# Autodesk Inventor assembly: 0008-10-10 Injectomat Standard
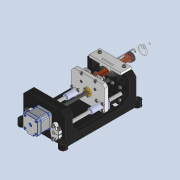
[picture p0: Inventor's stored thumbnail of the model, 180x180]
Saved by Autodesk Inventor 2020 (Build 240168000, 168)
## iProperties
Created: 2021-02-20
Part Number: 0008-10-10 Injectomat Standard
Document SubType Name: Assembly
Designer: Iulian Bors
Mass: 1274.49 g
Surface Area: 2683.15 cm^2
Volume: 830.675 cm^3
Density: 1.53428 g/cm^3
Description: Injectomat standard
Author: Iulian Bors
Subject: 10-10
## Documents named in this file (27)
- Z:\I.A.B\Proiecte\0008 I.A.B 3D 2.1 Imprimanta aracet Metal\10 Mecanic\0008-10-10 Injectomat Standard.iam
- Z:\I.A.B\Proiecte\0008 I.A.B 3D 2.1 Imprimanta aracet Metal\10 Mecanic\Seringa\syringe-57.snapshot.2\SYRINGE (INVENTOR)\Body Syringe.ipt
- Z:\I.A.B\Proiecte\0008 I.A.B 3D 2.1 Imprimanta aracet Metal\10 Mecanic\Seringa\syringe-57.snapshot.2\SYRINGE (INVENTOR)\Plunger.ipt
- Z:\I.A.B\Proiecte\0008 I.A.B 3D 2.1 Imprimanta aracet Metal\10 Mecanic\Seringa\syringe-57.snapshot.2\SYRINGE (INVENTOR)\Plunger Rubber.ipt
- Z:\I.A.B\Proiecte\0008 I.A.B 3D 2.1 Imprimanta aracet Metal\10 Mecanic\0008-10-1000 LMK8LUU.ipt
- Z:\I.A.B\Proiecte\0008 I.A.B 3D 2.1 Imprimanta aracet Metal\10 Mecanic\0008-10-1002  Hub.ipt
- Z:\I.A.B\Proiecte\0008 I.A.B 3D 2.1 Imprimanta aracet Metal\10 Mecanic\0008-10-1001 NEMA17 - Motor de passo.ipt
- Z:\I.A.B\Proiecte\0008 I.A.B 3D 2.1 Imprimanta aracet Metal\10 Mecanic\0008-10-1003 T8 screw.ipt
- Z:\I.A.B\Proiecte\0008 I.A.B 3D 2.1 Imprimanta aracet Metal\10 Mecanic\0008-10-001.ipt
- Z:\I.A.B\Proiecte\0008 I.A.B 3D 2.1 Imprimanta aracet Metal\10 Mecanic\0008-10-1005 ISO 1224-1 - 10 - 8 x 22 x 7.ipt
- Z:\I.A.B\Proiecte\0008 I.A.B 3D 2.1 Imprimanta aracet Metal\10 Mecanic\0008-10-002 Corp_Injectomat1.ipt
- Z:\I.A.B\Proiecte\0008 I.A.B 3D 2.1 Imprimanta aracet Metal\10 Mecanic\0008-10-1004 Piulita.ipt
- Z:\I.A.B\Proiecte\0008 I.A.B 3D 2.1 Imprimanta aracet Metal\10 Mecanic\0008-10-003.ipt
- Z:\I.A.B\Proiecte\0008 I.A.B 3D 2.1 Imprimanta aracet Metal\10 Mecanic\0008-10-1006 SHF8.ipt
- Z:\I.A.B\Proiecte\0008 I.A.B 3D 2.1 Imprimanta aracet Metal\10 Mecanic\0008-10-1007 Bara 8.ipt
- Z:\I.A.B\Proiecte\0008 I.A.B 3D 2.1 Imprimanta aracet Metal\10 Mecanic\0008-10-004 Fixare seringa.ipt
- Z:\I.A.B\Proiecte\0008 I.A.B 3D 2.1 Imprimanta aracet Metal\10 Mecanic\SurubM4x25.iam
- Z:\I.A.B\Proiecte\0008 I.A.B 3D 2.1 Imprimanta aracet Metal\10 Mecanic\SurubM4x35.iam
- Z:\I.A.B\Proiecte\0008 I.A.B 3D 2.1 Imprimanta aracet Metal\10 Mecanic\m3X16.iam
- Z:\I.A.B\Proiecte\0008 I.A.B 3D 2.1 Imprimanta aracet Metal\10 Mecanic\0008-10-2006 DIN 7984 - M3 x 16.ipt
- Z:\I.A.B\Proiecte\0008 I.A.B 3D 2.1 Imprimanta aracet Metal\10 Mecanic\0008-10-2007 DIN 7984 - M4 x 16.ipt
- Z:\I.A.B\Proiecte\0008 I.A.B 3D 2.1 Imprimanta aracet Metal\10 Mecanic\0008-10-2001 DIN 934 - M4 x 0.7.ipt
- Z:\I.A.B\Proiecte\0008 I.A.B 3D 2.1 Imprimanta aracet Metal\10 Mecanic\0008-10-005 Suport_Rulment.ipt
- Z:\I.A.B\Proiecte\0008 I.A.B 3D 2.1 Imprimanta aracet Metal\10 Mecanic\0008-10-2000 DIN 6912 - M4 x 25.ipt
- Z:\I.A.B\Proiecte\0008 I.A.B 3D 2.1 Imprimanta aracet Metal\10 Mecanic\0008-10-2008 DIN 912 - M3 x 0.5 x 25 x 18.ipt
- Z:\I.A.B\Proiecte\0008 I.A.B 3D 2.1 Imprimanta aracet Metal\10 Mecanic\0008-10-2005 DIN 125 - A 3.2.ipt
- Z:\I.A.B\Proiecte\0008 I.A.B 3D 2.1 Imprimanta aracet Metal\10 Mecanic\0008-10-2009 DIN 555-5 - M3.ipt
## Components (77 placed, 26 different names)
1. Body Syringe.ipt:1 — Mate:1, Mate:2, Mate:4, Tangent:1, Flush:5
2. Plunger.ipt:2 — Insert:1, Mate:3, Angle:6
3. Plunger Rubber.ipt:3 — Insert:1, Mate:1
4. 0008-10-1000 LMK8LUU.ipt:4 — Insert:6, Angle:5, Mate:13, Mate:17
5. 0008-10-1000 LMK8LUU.ipt:5 — Insert:5, Angle:4, Mate:12, Mate:15, Insert:30
6. 0008-10-1002  Hub.ipt:6 — Insert:2, Insert:3
7. 0008-10-1001 NEMA17 - Motor de passo.ipt:7 — Insert:3, Angle:2, Mate:4, Mate:5
8. 0008-10-1003 T8 screw.ipt:8 — Insert:2, Mate:21
9. 0008-10-001.ipt:9 — Angle:3, Mate:2, Mate:3, Flush:3, Insert:5, Angle:4, Insert:6, Angle:5, Mate:6, Mate:7, Insert:7, Mate:8, Mate:9, Mate:10
10. 0008-10-002 Corp_Injectomat1.ipt:10 — Mate:5, Mate:6, Mate:7, Tangent:1, Mate:11, Mate:14, Mate:16, Mate:18, Angle:7, Angle:9, Mate:19, Insert:32, Insert:44, Insert:48, Insert:49, Insert:50, Flush:6
11. 0008-10-1004 Piulita.ipt:11 — Insert:7, Insert:28, Mate:21
12. 0008-10-003.ipt:12 — Mate:8, Mate:9, Mate:10, Insert:23, Insert:24, Insert:25, Insert:26
13. 0008-10-1006 SHF8.ipt:13 — Mate:11, Mate:12, Insert:8, Angle:9, Insert:15, Insert:16, Insert:36
14. 0008-10-1007 Bara 8.ipt:14 — Insert:8
15. 0008-10-1007 Bara 8.ipt:15 — Insert:9
16. 0008-10-1006 SHF8.ipt:16 — Mate:13, Mate:14, Insert:9, Angle:10, Insert:17, Insert:18, Insert:38
17. 0008-10-1006 SHF8.ipt:17 — Mate:15, Mate:16, Angle:8, Insert:19, Insert:20, Insert:41
18. 0008-10-1006 SHF8.ipt:18 — Mate:17, Mate:18, Angle:7, Insert:21, Insert:22, Insert:42
19. 0008-10-004 Fixare seringa.ipt:19 — Mate:19, Flush:5, Insert:10, Insert:11, Flush:6
20. SurubM4x25.iam:20 [sub-assembly] — Insert:10
21. SurubM4x25.iam:21 [sub-assembly] — Insert:11
22. SurubM4x35.iam:22 [sub-assembly] — Insert:15
23. SurubM4x35.iam:23 [sub-assembly] — Insert:16
24. SurubM4x35.iam:24 [sub-assembly] — Insert:18
25. SurubM4x35.iam:25 [sub-assembly] — Insert:17
26. SurubM4x35.iam:26 [sub-assembly] — Insert:21
27. SurubM4x35.iam:27 [sub-assembly] — Insert:22
28. SurubM4x35.iam:28 [sub-assembly] — Insert:19
29. SurubM4x35.iam:29 [sub-assembly] — Insert:20
30. m3X16.iam:30 [sub-assembly] — Insert:23
31. m3X16.iam:31 [sub-assembly] — Insert:24
32. m3X16.iam:32 [sub-assembly] — Insert:25
33. m3X16.iam:33 [sub-assembly] — Insert:26
34. 0008-10-005 Suport_Rulment.ipt:58 — Insert:31, Angle:11, Insert:33, Insert:34
35. 0008-10-1005 ISO 1224-1 - 10 - 8 x 22 x 7.ipt:59 — Insert:31, Insert:32
36. SurubM4x35.iam:60 [sub-assembly] — Insert:34
37. SurubM4x35.iam:61 [sub-assembly] — Insert:33
38. 0008-10-2001 DIN 934 - M4 x 0.7.ipt:62 — Insert:35
39. 0008-10-2000 DIN 6912 - M4 x 25.ipt:63 — Insert:35, Insert:36
40. 0008-10-2001 DIN 934 - M4 x 0.7.ipt:64
41. 0008-10-2000 DIN 6912 - M4 x 25.ipt:65 — Insert:38
42. 0008-10-2001 DIN 934 - M4 x 0.7.ipt:66
43. 0008-10-2000 DIN 6912 - M4 x 25.ipt:67 — Insert:41
44. 0008-10-2001 DIN 934 - M4 x 0.7.ipt:68
45. 0008-10-2000 DIN 6912 - M4 x 25.ipt:69 — Insert:42
46. 0008-10-2008 DIN 912 - M3 x 0.5 x 25 x 18.ipt:70 — Insert:43
47. 0008-10-2005 DIN 125 - A 3.2.ipt:71 — Insert:43, Insert:44
48. 0008-10-2008 DIN 912 - M3 x 0.5 x 25 x 18.ipt:72
49. 0008-10-2005 DIN 125 - A 3.2.ipt:73 — Insert:50
50. 0008-10-2008 DIN 912 - M3 x 0.5 x 25 x 18.ipt:74
51. 0008-10-2005 DIN 125 - A 3.2.ipt:75 — Insert:48
52. 0008-10-2008 DIN 912 - M3 x 0.5 x 25 x 18.ipt:76
53. 0008-10-2005 DIN 125 - A 3.2.ipt:77 — Insert:49
54. 0008-10-2006 DIN 7984 - M3 x 16.ipt:34 — Insert:27, Insert:28
55. 0008-10-2009 DIN 555-5 - M3.ipt:35 — Insert:27
56. 0008-10-2006 DIN 7984 - M3 x 16.ipt:36
57. 0008-10-2009 DIN 555-5 - M3.ipt:37
58. 0008-10-2006 DIN 7984 - M3 x 16.ipt:38
59. 0008-10-2009 DIN 555-5 - M3.ipt:39
60. 0008-10-2006 DIN 7984 - M3 x 16.ipt:40
61. 0008-10-2009 DIN 555-5 - M3.ipt:41
62. 0008-10-2001 DIN 934 - M4 x 0.7.ipt:42 — Insert:29
63. 0008-10-2007 DIN 7984 - M4 x 16.ipt:43 — Insert:29, Insert:30
64. 0008-10-2001 DIN 934 - M4 x 0.7.ipt:44
65. 0008-10-2007 DIN 7984 - M4 x 16.ipt:45
66. 0008-10-2001 DIN 934 - M4 x 0.7.ipt:46
67. 0008-10-2007 DIN 7984 - M4 x 16.ipt:47
68. 0008-10-2001 DIN 934 - M4 x 0.7.ipt:48
69. 0008-10-2007 DIN 7984 - M4 x 16.ipt:49
70. 0008-10-2001 DIN 934 - M4 x 0.7.ipt:50
71. 0008-10-2007 DIN 7984 - M4 x 16.ipt:51
72. 0008-10-2001 DIN 934 - M4 x 0.7.ipt:52
73. 0008-10-2007 DIN 7984 - M4 x 16.ipt:53
74. 0008-10-2001 DIN 934 - M4 x 0.7.ipt:54
75. 0008-10-2007 DIN 7984 - M4 x 16.ipt:55
76. 0008-10-2001 DIN 934 - M4 x 0.7.ipt:56
77. 0008-10-2007 DIN 7984 - M4 x 16.ipt:57
## Component patterns: (4 elements, first: 0008-10-2006 DIN 7984 - M3 x 16.ipt:34 + 0008-10-2009 DIN 555-5 - M3.ipt:35), (2 elements), (4 elements, first: 0008-10-2001 DIN 934 - M4 x 0.7.ipt:42 + 0008-10-2007 DIN 7984 - M4 x 16.ipt:43), Component Pattern 2:2 (4 elements)
## Relationships (80: Insert 46, Mate 20, Angle 10, Flush 3, Tangent 1)
- Insert:1: Plunger.ipt:2 ↔ Plunger Rubber.ipt:3
- Mate:1: Body Syringe.ipt:1 ↔ Plunger Rubber.ipt:3
- Insert:2: 0008-10-1002  Hub.ipt:6 ↔ 0008-10-1003 T8 screw.ipt:8
- Insert:3: 0008-10-1002  Hub.ipt:6 ↔ 0008-10-1001 NEMA17 - Motor de passo.ipt:7
- Angle:2 (0 deg): 0008-10-1001 NEMA17 - Motor de passo.ipt:7
- Angle:3 (0 deg): 0008-10-001.ipt:9
- Mate:2: Body Syringe.ipt:1 ↔ 0008-10-001.ipt:9
- Mate:3: Plunger.ipt:2 ↔ 0008-10-001.ipt:9
- Flush:3 (-13.343 mm): 0008-10-001.ipt:9
- Mate:4: Body Syringe.ipt:1 ↔ 0008-10-1001 NEMA17 - Motor de passo.ipt:7
- Insert:5: 0008-10-1000 LMK8LUU.ipt:5 ↔ 0008-10-001.ipt:9
- Angle:4 (0 deg): 0008-10-1000 LMK8LUU.ipt:5 ↔ 0008-10-001.ipt:9
- Insert:6: 0008-10-1000 LMK8LUU.ipt:4 ↔ 0008-10-001.ipt:9
- Angle:5 (0 deg): 0008-10-1000 LMK8LUU.ipt:4 ↔ 0008-10-001.ipt:9
- Mate:5: 0008-10-1001 NEMA17 - Motor de passo.ipt:7 ↔ 0008-10-002 Corp_Injectomat1.ipt:10
- Mate:6: 0008-10-001.ipt:9 ↔ 0008-10-002 Corp_Injectomat1.ipt:10
- Mate:7 (5 mm): 0008-10-001.ipt:9 ↔ 0008-10-002 Corp_Injectomat1.ipt:10
- Insert:7: 0008-10-001.ipt:9 ↔ 0008-10-1004 Piulita.ipt:11
- Mate:8: 0008-10-001.ipt:9 ↔ 0008-10-003.ipt:12
- Mate:9 (-27 mm): 0008-10-001.ipt:9 ↔ 0008-10-003.ipt:12
- Mate:10: 0008-10-001.ipt:9 ↔ 0008-10-003.ipt:12
- Angle:6 (0 deg): Plunger.ipt:2
- Tangent:1: Body Syringe.ipt:1 ↔ 0008-10-002 Corp_Injectomat1.ipt:10
- Mate:11: 0008-10-002 Corp_Injectomat1.ipt:10 ↔ 0008-10-1006 SHF8.ipt:13
- Mate:12: 0008-10-1000 LMK8LUU.ipt:5 ↔ 0008-10-1006 SHF8.ipt:13
- Insert:8: 0008-10-1006 SHF8.ipt:13 ↔ 0008-10-1007 Bara 8.ipt:14
- Mate:13: 0008-10-1000 LMK8LUU.ipt:4 ↔ 0008-10-1006 SHF8.ipt:16
- Mate:14: 0008-10-002 Corp_Injectomat1.ipt:10 ↔ 0008-10-1006 SHF8.ipt:16
- Mate:15: 0008-10-1000 LMK8LUU.ipt:5 ↔ 0008-10-1006 SHF8.ipt:17
- Mate:16: 0008-10-002 Corp_Injectomat1.ipt:10 ↔ 0008-10-1006 SHF8.ipt:17
- Mate:17: 0008-10-1000 LMK8LUU.ipt:4 ↔ 0008-10-1006 SHF8.ipt:18
- Mate:18: 0008-10-002 Corp_Injectomat1.ipt:10 ↔ 0008-10-1006 SHF8.ipt:18
- Insert:9: 0008-10-1007 Bara 8.ipt:15 ↔ 0008-10-1006 SHF8.ipt:16
- Angle:7 (0 deg): 0008-10-002 Corp_Injectomat1.ipt:10 ↔ 0008-10-1006 SHF8.ipt:18
- Angle:8 (180 deg): 0008-10-1006 SHF8.ipt:17
- Angle:9 (0 deg): 0008-10-002 Corp_Injectomat1.ipt:10 ↔ 0008-10-1006 SHF8.ipt:13
- Angle:10 (0 deg): 0008-10-1006 SHF8.ipt:16
- Mate:19 (-6 mm): 0008-10-002 Corp_Injectomat1.ipt:10 ↔ 0008-10-004 Fixare seringa.ipt:19
- Flush:5: Body Syringe.ipt:1 ↔ 0008-10-004 Fixare seringa.ipt:19
- Insert:10: 0008-10-004 Fixare seringa.ipt:19 ↔ SurubM4x25.iam:20
- Insert:11: 0008-10-004 Fixare seringa.ipt:19 ↔ SurubM4x25.iam:21
- Insert:15: 0008-10-1006 SHF8.ipt:13 ↔ SurubM4x35.iam:22
- Insert:16: 0008-10-1006 SHF8.ipt:13 ↔ SurubM4x35.iam:23
- Insert:17: 0008-10-1006 SHF8.ipt:16 ↔ SurubM4x35.iam:25
- Insert:18: 0008-10-1006 SHF8.ipt:16 ↔ SurubM4x35.iam:24
- Insert:19: 0008-10-1006 SHF8.ipt:17 ↔ SurubM4x35.iam:28
- Insert:20: 0008-10-1006 SHF8.ipt:17 ↔ SurubM4x35.iam:29
- Insert:21: 0008-10-1006 SHF8.ipt:18 ↔ SurubM4x35.iam:26
- Insert:22: 0008-10-1006 SHF8.ipt:18 ↔ SurubM4x35.iam:27
- Insert:23: 0008-10-003.ipt:12 ↔ m3X16.iam:30
- Insert:24: 0008-10-003.ipt:12 ↔ m3X16.iam:31
- Insert:25: 0008-10-003.ipt:12 ↔ m3X16.iam:32
- Insert:26: 0008-10-003.ipt:12 ↔ m3X16.iam:33
- Insert:27: 0008-10-2006 DIN 7984 - M3 x 16.ipt:34 ↔ 0008-10-2009 DIN 555-5 - M3.ipt:35
- Insert:28: 0008-10-1004 Piulita.ipt:11 ↔ 0008-10-2006 DIN 7984 - M3 x 16.ipt:34
- Insert:29: 0008-10-2001 DIN 934 - M4 x 0.7.ipt:42 ↔ 0008-10-2007 DIN 7984 - M4 x 16.ipt:43
- Insert:30: 0008-10-1000 LMK8LUU.ipt:5 ↔ 0008-10-2007 DIN 7984 - M4 x 16.ipt:43
- Mate:21: 0008-10-1003 T8 screw.ipt:8 ↔ 0008-10-1004 Piulita.ipt:11
- Insert:31: 0008-10-005 Suport_Rulment.ipt:58 ↔ 0008-10-1005 ISO 1224-1 - 10 - 8 x 22 x 7.ipt:59
- Insert:32: 0008-10-002 Corp_Injectomat1.ipt:10 ↔ 0008-10-1005 ISO 1224-1 - 10 - 8 x 22 x 7.ipt:59
- Angle:11 (0 deg): 0008-10-005 Suport_Rulment.ipt:58
- Insert:33: 0008-10-005 Suport_Rulment.ipt:58 ↔ SurubM4x35.iam:61
- Insert:34: 0008-10-005 Suport_Rulment.ipt:58 ↔ SurubM4x35.iam:60
- Insert:35: 0008-10-2001 DIN 934 - M4 x 0.7.ipt:62 ↔ 0008-10-2000 DIN 6912 - M4 x 25.ipt:63
- Insert:36: 0008-10-1006 SHF8.ipt:13 ↔ 0008-10-2000 DIN 6912 - M4 x 25.ipt:63
- [Insert]: 0008-10-2001 DIN 934 - M4 x 0.7.ipt:64 ↔ 0008-10-2000 DIN 6912 - M4 x 25.ipt:65
- Insert:38: 0008-10-1006 SHF8.ipt:16 ↔ 0008-10-2000 DIN 6912 - M4 x 25.ipt:65
- [Insert]: 0008-10-2001 DIN 934 - M4 x 0.7.ipt:66 ↔ 0008-10-2000 DIN 6912 - M4 x 25.ipt:67
- [Insert]: 0008-10-2001 DIN 934 - M4 x 0.7.ipt:68 ↔ 0008-10-2000 DIN 6912 - M4 x 25.ipt:69
- Insert:41: 0008-10-1006 SHF8.ipt:17 ↔ 0008-10-2000 DIN 6912 - M4 x 25.ipt:67
- Insert:42: 0008-10-1006 SHF8.ipt:18 ↔ 0008-10-2000 DIN 6912 - M4 x 25.ipt:69
- Insert:43: 0008-10-2008 DIN 912 - M3 x 0.5 x 25 x 18.ipt:70 ↔ 0008-10-2005 DIN 125 - A 3.2.ipt:71
- Insert:44: 0008-10-002 Corp_Injectomat1.ipt:10 ↔ 0008-10-2005 DIN 125 - A 3.2.ipt:71
- [Insert]: 0008-10-2008 DIN 912 - M3 x 0.5 x 25 x 18.ipt:72 ↔ 0008-10-2005 DIN 125 - A 3.2.ipt:73
- [Insert]: 0008-10-2008 DIN 912 - M3 x 0.5 x 25 x 18.ipt:74 ↔ 0008-10-2005 DIN 125 - A 3.2.ipt:75
- [Insert]: 0008-10-2008 DIN 912 - M3 x 0.5 x 25 x 18.ipt:76 ↔ 0008-10-2005 DIN 125 - A 3.2.ipt:77
- Insert:48: 0008-10-002 Corp_Injectomat1.ipt:10 ↔ 0008-10-2005 DIN 125 - A 3.2.ipt:75
- Insert:49: 0008-10-002 Corp_Injectomat1.ipt:10 ↔ 0008-10-2005 DIN 125 - A 3.2.ipt:77
- Insert:50: 0008-10-002 Corp_Injectomat1.ipt:10 ↔ 0008-10-2005 DIN 125 - A 3.2.ipt:73
- Flush:6 (-0.25 mm): 0008-10-002 Corp_Injectomat1.ipt:10 ↔ 0008-10-004 Fixare seringa.ipt:19
## Named parameters: d90_d88 = 0 mm, d92_d88 = 0 mm, d93_d88 = 0 mm, d98_d96 = 0 mm, d99_d96 = 0 mm, d100_d96 = 0 mm
